# Autodesk Inventor assembly: Assembly1
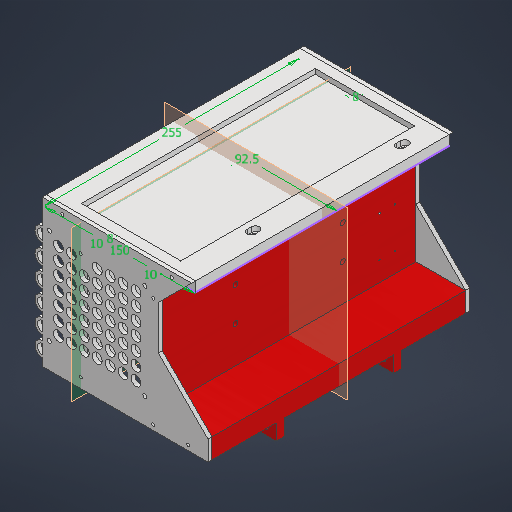
[picture p0: Inventor's stored thumbnail of the model, 512x512]
Saved by Autodesk Inventor 2025.1 (Build 291241000, 241)
## iProperties
Created: 2025-03-19
Part Number: Assembly1
Document SubType Name: Assembly
Designer: m_kni
Author: m_kni
## Documents named in this file (6)
- C:\Users\jerem\Documents\GitHub\Perovskite-Automated-Synthesis-System\CAD\Ebox\Assembly1.iam
- C:\Users\jerem\Documents\GitHub\Perovskite-Automated-Synthesis-System\CAD\Ebox\EboxCase.ipt
- C:\Users\jerem\Documents\GitHub\Perovskite-Automated-Synthesis-System\CAD\Ebox\SidePlate_Ebox.ipt
- C:\Users\jerem\Documents\GitHub\Perovskite-Automated-Synthesis-System\CAD\Ebox\bottomplate.ipt
- C:\Users\jerem\Documents\GitHub\Perovskite-Automated-Synthesis-System\CAD\Ebox\midplate.ipt
- C:\Users\jerem\Documents\GitHub\Perovskite-Automated-Synthesis-System\CAD\Ebox\PSU.ipt
## Components (6 placed, 5 different names)
1. EboxCase:1 — Insert:1, Flush:1, Insert:2, Flush:2, Mate:1
2. SidePlate_Ebox:1 — Insert:1, Flush:1, Insert:3, Insert:4, Angle:1
3. SidePlate_Ebox:2 — Insert:2, Flush:2
4. bottomplate:1 — Insert:3
5. midplate:1 — Insert:4, Angle:1
6. PSU:1 — Mate:1
## Relationships (8: Insert 4, Flush 2, Angle 1, Mate 1)
- Insert:1: EboxCase:1 ↔ SidePlate_Ebox:1
- Flush:1: EboxCase:1 ↔ SidePlate_Ebox:1
- Insert:2: EboxCase:1 ↔ SidePlate_Ebox:2
- Flush:2: EboxCase:1 ↔ SidePlate_Ebox:2
- Insert:3: SidePlate_Ebox:1 ↔ bottomplate:1
- Insert:4: SidePlate_Ebox:1 ↔ midplate:1
- Angle:1 (0 deg): SidePlate_Ebox:1 ↔ midplate:1
- Mate:1: EboxCase:1 ↔ PSU:1
